# Autodesk Inventor assembly: Kornylak Wheel
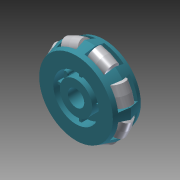
[picture p0: Inventor's stored thumbnail of the model, 180x180]
Saved by Autodesk Inventor 2014 (Build 180170000, 170)
## iProperties
Created: 2014-02-14
Part Number: Kornylak Wheel
Document SubType Name: Assembly
Designer: Spooner
Author: Spooner
## Documents named in this file (3)
- C:\Users\Spooner\Documents\Inventor\FerretBall Robot\3Pod\Inventor 2014 Files\Kornylak Wheel.iam
- C:\Users\Spooner\Documents\Inventor\FerretBall Robot\3Pod\Inventor 2014 Files\Kornylak- Half Wheel.ipt
- C:\Users\Spooner\Documents\Inventor\FerretBall Robot\3Pod\Inventor 2014 Files\Kornylak- Roller.ipt
## Components (10 placed, 2 different names)
1. Kornylak- Half Wheel:1 — Insert:1, Insert:2, Insert:3, Insert:4, Insert:5, Insert:6, Insert:7, Insert:8, Insert:9, Angle:1
2. Kornylak- Half Wheel:2 — Insert:9, Angle:1
3. Kornylak- Roller:1 — Insert:1
4. Kornylak- Roller:2 — Insert:2
5. Kornylak- Roller:3 — Insert:3
6. Kornylak- Roller:4 — Insert:4
7. Kornylak- Roller:5 — Insert:5
8. Kornylak- Roller:6 — Insert:6
9. Kornylak- Roller:7 — Insert:7
10. Kornylak- Roller:8 — Insert:8
## Relationships (10: Insert 9, Angle 1)
- Insert:1: Kornylak- Half Wheel:1 ↔ Kornylak- Roller:1
- Insert:2: Kornylak- Half Wheel:1 ↔ Kornylak- Roller:2
- Insert:3: Kornylak- Half Wheel:1 ↔ Kornylak- Roller:3
- Insert:4: Kornylak- Half Wheel:1 ↔ Kornylak- Roller:4
- Insert:5: Kornylak- Half Wheel:1 ↔ Kornylak- Roller:5
- Insert:6: Kornylak- Half Wheel:1 ↔ Kornylak- Roller:6
- Insert:7: Kornylak- Half Wheel:1 ↔ Kornylak- Roller:7
- Insert:8: Kornylak- Half Wheel:1 ↔ Kornylak- Roller:8
- Insert:9: Kornylak- Half Wheel:1 ↔ Kornylak- Half Wheel:2
- Angle:1 (180 deg): Kornylak- Half Wheel:1 ↔ Kornylak- Half Wheel:2
